# Autodesk Inventor assembly: LiftAssembly_Through
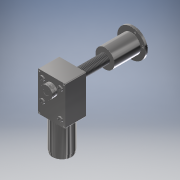
[picture p0: Inventor's stored thumbnail of the model, 180x180]
Saved by Autodesk Inventor 2018 (Build 220112000, 112)
## iProperties
Created: 2018-04-10
Part Number: LiftAssembly_Through
Document SubType Name: Assembly
Designer: P136265
Author: P136265
## Documents named in this file (6)
- C:\Users\P136265\Documents\GitHub\mecanum-cad\LiftAssembly_Through.iam
- C:\Users\P136265\Documents\GitHub\mecanum-cad\LeadScrew.ipt
- C:\Users\P136265\Documents\GitHub\mecanum-cad\TS-58GZ868D_Open.ipt
- C:\Users\P136265\Documents\GitHub\mecanum-cad\RNFBL2005A2.5S.ipt
- C:\Users\P136265\Documents\Inventor\Content Center Files\R2018\en-US\ISO 3031(1)\ISO 3031 - 12 x 26 x 2(1).ipt
- C:\Users\P136265\Documents\GitHub\mecanum-cad\ThrustWasher.ipt
## Components (6 placed, 5 different names)
1. TS-58GZ868D_Open:1 — Mate:5, Mate:8, Mate:13, Mate:14, Angle:2, Mate:16
2. LeadScrew:2 — Mate:5, Mate:8, Mate:12, Mate:18, Mate:19, Mate:20
3. RNFBL2005A2.5S:2 — Mate:12, Mate:13
4. ISO 3031Thrust Needle Roller And Cage Assembly 12 x 26 x 2:1 — Mate:18, Mate:21, Mate:22, Mate:23
5. ThrustWasher:1 — Mate:22, Mate:23
6. ThrustWasher:2 — Mate:19, Mate:20, Mate:21
## Relationships (13: Mate 12, Angle 1)
- Mate:5: TS-58GZ868D_Open:1 ↔ LeadScrew:2
- Mate:8: TS-58GZ868D_Open:1 ↔ LeadScrew:2
- Mate:12: LeadScrew:2 ↔ RNFBL2005A2.5S:2
- Mate:13: TS-58GZ868D_Open:1 ↔ RNFBL2005A2.5S:2
- Mate:14: TS-58GZ868D_Open:1
- Angle:2 (0 deg): TS-58GZ868D_Open:1
- Mate:16: TS-58GZ868D_Open:1
- Mate:18: LeadScrew:2 ↔ ISO 3031Thrust Needle Roller And Cage Assembly 12 x 26 x 2:1
- Mate:19: LeadScrew:2 ↔ ThrustWasher:2
- Mate:20: LeadScrew:2 ↔ ThrustWasher:2
- Mate:21 (0.2 mm): ISO 3031Thrust Needle Roller And Cage Assembly 12 x 26 x 2:1 ↔ ThrustWasher:2
- Mate:22: ISO 3031Thrust Needle Roller And Cage Assembly 12 x 26 x 2:1 ↔ ThrustWasher:1
- Mate:23 (0.2 mm): ISO 3031Thrust Needle Roller And Cage Assembly 12 x 26 x 2:1 ↔ ThrustWasher:1
